# Autodesk Inventor assembly: Assembly1
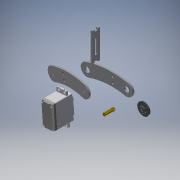
[picture p0: Inventor's stored thumbnail of the model, 180x180]
Saved by Autodesk Inventor 2019 (Build 230136000, 136)
## iProperties
Created: 2023-04-16
Part Number: Assembly1
Document SubType Name: Assembly
Designer: Analuam
Author: Analuam
## Documents named in this file (9)
- D:\Assembly1.iam
- D:\Dek Diyah\fem.ipt
- D:\Dek Diyah\servomg996r\Acople circular.ipt
- D:\Dek Diyah\servomg996r\Base.ipt
- D:\Dek Diyah\servomg996r\Eje.ipt
- D:\Dek Diyah\servomg996r\Medio.ipt
- D:\Dek Diyah\servomg996r\Top.ipt
- D:\Dek Diyah\fem2.ipt
- D:\Dek Diyah\HubFem.ipt
## Components (8 placed, 8 different names)
1. fem:1
2. Acople circular:1
3. Base:1 — Flush:4, Flush:5, Mate:5
4. Eje:1
5. Medio:1 — Flush:2, Flush:3, Mate:4, Flush:4, Flush:5, Mate:5
6. Top:1 — Flush:2, Flush:3, Mate:4
7. fem2:1
8. HubFem:1
## Relationships (6: Flush 4, Mate 2)
- Flush:2: Medio:1 ↔ Top:1
- Flush:3: Medio:1 ↔ Top:1
- Mate:4: Medio:1 ↔ Top:1
- Flush:4: Base:1 ↔ Medio:1
- Flush:5: Base:1 ↔ Medio:1
- Mate:5: Base:1 ↔ Medio:1
